# Autodesk Inventor assembly: B Idler
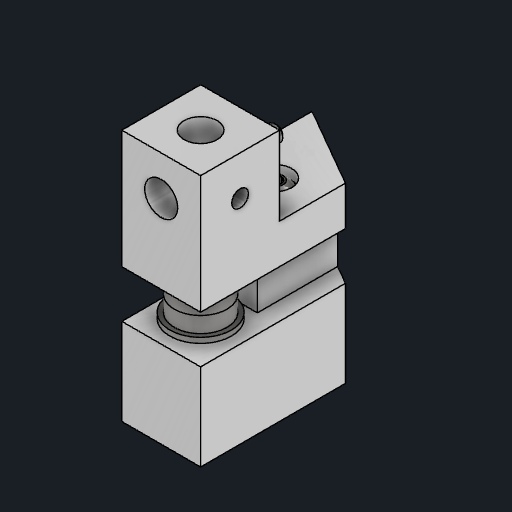
[picture p0: Inventor's stored thumbnail of the model, 512x512]
Saved by Autodesk Inventor 2026 (Build 300175050, 175E)
## iProperties
Created: 2025-05-09
Part Number: B Idler
Document SubType Name: Assembly
Designer: AdminForWorker
Title: B Idler
Author: AdminForWorker
## Documents named in this file (6)
- C:\Users\Joshua Eah\Documents\GitHub\Voron-0\CAD\Master Assembly\Idlers\B Idler.iam
- C:\Users\Joshua Eah\Documents\GitHub\Voron-0\CAD\Machined Parts\Idlers\B Idler\B Idler.ipt
- C:\Users\Joshua Eah\Documents\GitHub\Voron-0\CAD\Master Assembly\Hardware\M3 Hexnut.ipt
- C:\Users\Joshua Eah\Documents\GitHub\Voron-0\CAD\Master Assembly\Hardware\F623 Stack.iam
- C:\Users\Joshua Eah\Documents\GitHub\Voron-0\CAD\Master Assembly\Hardware\M3x10 BHCS.ipt
- C:\Users\Joshua Eah\Documents\GitHub\Voron-0\CAD\Master Assembly\Hardware\M3x35 BHCS.ipt
## Components (6 placed, 5 different names)
1. B Idler:1
2. M3 Hexnut:1
3. F623 Stack:1 [sub-assembly]
4. M3x10 BHCS:1
5. M3x35 BHCS:1
6. M3x35 BHCS:2
## Relationships (1: Insert 1)
- [Insert]: B Idler:1 ↔ M3x10 BHCS:1
